# Autodesk Inventor assembly: CompleteSocket
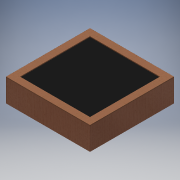
[picture p0: Inventor's stored thumbnail of the model, 180x180]
Saved by Autodesk Inventor 2019.3 (Build 233278000, 278)
## iProperties
Created: 2019-01-12
Part Number: CompleteSocket
Material: Generisch
Document SubType Name: Assembly
Designer: Jonas
Author: Jonas
## Documents named in this file (13)
- C:\Users\Jonas\Desktop\RGBCube-v2\CAD\Socket\CompleteSocket.iam
- C:\Users\Jonas\Desktop\RGBCube-v2\CAD\Socket\WoodenSocket.iam
- C:\Users\Jonas\Desktop\RGBCube-v2\CAD\Socket\Cover.ipt
- C:\Users\Jonas\Desktop\RGBCube-v2\CAD\Socket\Spacer.ipt
- C:\Users\Jonas\Desktop\RGBCube-v2\CAD\Socket\CompleteSocket\Konstruktions-Assistent\Schraubenverbindung2.iam
- C:\Users\Jonas\Desktop\RGBCube-v2\CAD\Socket\CompleteSocket\Konstruktions-Assistent\Schraubenverbindung3.iam
- C:\Users\Jonas\Desktop\RGBCube-v2\CAD\Socket\CompleteSocket\Konstruktions-Assistent\Schraubenverbindung4.iam
- C:\Users\Jonas\Desktop\RGBCube-v2\CAD\Socket\CompleteSocket\Konstruktions-Assistent\Schraubenverbindung5.iam
- C:\Users\Jonas\Desktop\RGBCube-v2\CAD\Socket\CompleteSocket\Konstruktions-Assistent\Schraubenverbindung6.iam
- C:\Users\Jonas\Desktop\RGBCube-v2\CAD\Socket\CompleteSocket\Konstruktions-Assistent\Schraubenverbindung7.iam
- C:\Users\Jonas\Desktop\RGBCube-v2\CAD\Socket\CompleteSocket\Konstruktions-Assistent\Schraubenverbindung8.iam
- C:\Users\Jonas\Desktop\RGBCube-v2\CAD\Socket\CompleteSocket\Konstruktions-Assistent\Schraubenverbindung9.iam
- C:\Users\Jonas\Desktop\RGBCube-v2\CAD\Socket\EdgeCover.ipt
## Components (18 placed, 5 different names)
1. WoodenSocket:1 [sub-assembly] — Passend:1, Passend:2, Passend:3, Passend:5, Passend:6, Passend:8, Passend:9, Passend:11, Passend:12, Passend:14, Passend:31, Passend:32, Fluchtend:1, Passend:33, Fluchtend:2, Passend:34, Passend:35, Fluchtend:3, Passend:36, Fluchtend:4, Passend:37, Passend:38
2. Cover:1 — Passend:1, Passend:2, Passend:4, Passend:7, Passend:10, Passend:13
3. Spacer:1 — Passend:3, Passend:4, Passend:5, Passend:23, Passend:24, Passend:25, Passend:26
4. Spacer:2 — Passend:6, Passend:7, Passend:8, Passend:27, Passend:28, Passend:29, Passend:30
5. Spacer:3 — Passend:9, Passend:10, Passend:11, Passend:15, Passend:16, Passend:17, Passend:18
6. Spacer:4 — Passend:12, Passend:13, Passend:14, Passend:19, Passend:20, Passend:21, Passend:22
7. Schraubenverbindung:1 [sub-assembly] — Passend:15, Passend:16
8. Schraubenverbindung:2 [sub-assembly] — Passend:17, Passend:18
9. Schraubenverbindung:3 [sub-assembly] — Passend:19, Passend:20
10. Schraubenverbindung:4 [sub-assembly] — Passend:21, Passend:22
11. Schraubenverbindung:5 [sub-assembly] — Passend:23, Passend:24
12. Schraubenverbindung:6 [sub-assembly] — Passend:25, Passend:26
13. Schraubenverbindung:7 [sub-assembly] — Passend:27, Passend:28
14. Schraubenverbindung:8 [sub-assembly] — Passend:29, Passend:30
15. EdgeCover:1 — Passend:31, Passend:32, Fluchtend:1
16. EdgeCover:2 — Passend:33, Fluchtend:2, Passend:34
17. EdgeCover:3 — Passend:35, Fluchtend:3, Passend:36
18. EdgeCover:4 — Fluchtend:4, Passend:37, Passend:38
## Relationships (42: Mate 38, Flush 4)
- Passend:1 [Mate]: WoodenSocket:1 ↔ Cover:1
- Passend:2 [Mate]: WoodenSocket:1 ↔ Cover:1
- Passend:3 [Mate]: WoodenSocket:1 ↔ Spacer:1
- Passend:4 [Mate]: Cover:1 ↔ Spacer:1
- Passend:5 [Mate] (12 mm): WoodenSocket:1 ↔ Spacer:1
- Passend:6 [Mate]: WoodenSocket:1 ↔ Spacer:2
- Passend:7 [Mate]: Cover:1 ↔ Spacer:2
- Passend:8 [Mate] (12 mm): WoodenSocket:1 ↔ Spacer:2
- Passend:9 [Mate]: WoodenSocket:1 ↔ Spacer:3
- Passend:10 [Mate]: Cover:1 ↔ Spacer:3
- Passend:11 [Mate] (12 mm): WoodenSocket:1 ↔ Spacer:3
- Passend:12 [Mate]: WoodenSocket:1 ↔ Spacer:4
- Passend:13 [Mate]: Cover:1 ↔ Spacer:4
- Passend:14 [Mate] (12 mm): WoodenSocket:1 ↔ Spacer:4
- Passend:15 [Mate]: Spacer:3 ↔ Schraubenverbindung:1
- Passend:16 [Mate]: Spacer:3 ↔ Schraubenverbindung:1
- Passend:17 [Mate]: Spacer:3 ↔ Schraubenverbindung:2
- Passend:18 [Mate]: Spacer:3 ↔ Schraubenverbindung:2
- Passend:19 [Mate]: Spacer:4 ↔ Schraubenverbindung:3
- Passend:20 [Mate]: Spacer:4 ↔ Schraubenverbindung:3
- Passend:21 [Mate]: Spacer:4 ↔ Schraubenverbindung:4
- Passend:22 [Mate]: Spacer:4 ↔ Schraubenverbindung:4
- Passend:23 [Mate]: Spacer:1 ↔ Schraubenverbindung:5
- Passend:24 [Mate]: Spacer:1 ↔ Schraubenverbindung:5
- Passend:25 [Mate]: Spacer:1 ↔ Schraubenverbindung:6
- Passend:26 [Mate]: Spacer:1 ↔ Schraubenverbindung:6
- Passend:27 [Mate]: Spacer:2 ↔ Schraubenverbindung:7
- Passend:28 [Mate]: Spacer:2 ↔ Schraubenverbindung:7
- Passend:29 [Mate]: Spacer:2 ↔ Schraubenverbindung:8
- Passend:30 [Mate]: Spacer:2 ↔ Schraubenverbindung:8
- Passend:31 [Mate]: WoodenSocket:1 ↔ EdgeCover:1
- Passend:32 [Mate]: WoodenSocket:1 ↔ EdgeCover:1
- Fluchtend:1 [Flush]: WoodenSocket:1 ↔ EdgeCover:1
- Passend:33 [Mate]: WoodenSocket:1 ↔ EdgeCover:2
- Fluchtend:2 [Flush]: WoodenSocket:1 ↔ EdgeCover:2
- Passend:34 [Mate]: WoodenSocket:1 ↔ EdgeCover:2
- Passend:35 [Mate]: WoodenSocket:1 ↔ EdgeCover:3
- Fluchtend:3 [Flush]: WoodenSocket:1 ↔ EdgeCover:3
- Passend:36 [Mate]: WoodenSocket:1 ↔ EdgeCover:3
- Fluchtend:4 [Flush]: WoodenSocket:1 ↔ EdgeCover:4
- Passend:37 [Mate]: WoodenSocket:1 ↔ EdgeCover:4
- Passend:38 [Mate]: WoodenSocket:1 ↔ EdgeCover:4
